# Autodesk Inventor assembly: walle_s_cinkou
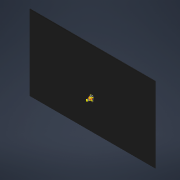
[picture p0: Inventor's stored thumbnail of the model, 180x180]
Saved by Autodesk Inventor 2022 (Build 260153000, 153)
## iProperties
Created: 2022-02-12
Part Number: walle_s_cinkou
Document SubType Name: Assembly
Designer: Lukas
Author: Lukas
## Documents named in this file (4)
- C:\Users\Lukas\Desktop\ard\3D\Walle\FINAL\assembly\walle_s_cinkou.iam
- C:\Users\Lukas\Desktop\ard\3D\Walle\FINAL\assembly\McCrea_WALLE_bez_HEAD_walle.iam
- C:\Users\Lukas\Desktop\ard\3D\Walle\FINAL\lukas\McCrea_cinka_walle.ipt
- C:\Users\Lukas\Desktop\ard\3D\Walle\FINAL\matus\plocha\McCrea_plocha_walle.ipt
## Components (4 placed, 3 different names)
1. McCrea_WALLE_bez_HEAD_walle:1 [sub-assembly] — Mate:1, Mate:2
2. McCrea_cinka_walle:1 — Mate:1
3. McCrea_cinka_walle:2 — Mate:2
4. McCrea_plocha_walle:1
## Relationships (2: Mate 2)
- Mate:1: McCrea_WALLE_bez_HEAD_walle:1 ↔ McCrea_cinka_walle:1
- Mate:2: McCrea_WALLE_bez_HEAD_walle:1 ↔ McCrea_cinka_walle:2
